# Autodesk Inventor assembly: Ortak
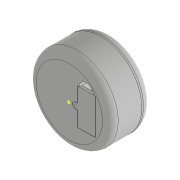
[picture p0: Inventor's stored thumbnail of the model, 180x180]
Saved by Autodesk Inventor 2022 (Build 260153000, 153)
## iProperties
Created: 2023-02-07
Part Number: Ortak
Document SubType Name: Assembly
Designer: MVeszpremi
Author: MVeszpremi
## Documents named in this file (4)
- C:\Users\veszp\Dropbox\180DAB CAD\Ortak.iam
- C:\Users\veszp\Dropbox\180DAB CAD\OrTak.ipt
- C:\Users\veszp\Dropbox\180DAB CAD\OrTak_lod.ipt
- C:\Users\veszp\Dropbox\180DAB CAD\Ortak_bat_lid.ipt
## Components (3 placed, 3 different names)
1. OrTak:1 — Mate:1, Mate:2, Mate:3, Mate:4, Mate:5
2. OrTak_lod:1 — Mate:1, Mate:2, Mate:3
3. Ortak_bat_lid:1 — Mate:4, Mate:5
## Relationships (5: Mate 5)
- Mate:1: OrTak:1 ↔ OrTak_lod:1
- Mate:2: OrTak:1 ↔ OrTak_lod:1
- Mate:3: OrTak:1 ↔ OrTak_lod:1
- Mate:4: OrTak:1 ↔ Ortak_bat_lid:1
- Mate:5: OrTak:1 ↔ Ortak_bat_lid:1
